# Autodesk Inventor assembly: y-axis
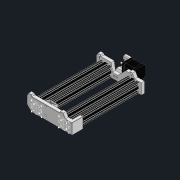
[picture p0: Inventor's stored thumbnail of the model, 180x180]
Saved by Autodesk Inventor 2021 (Build 250183000, 183)
## iProperties
Created: 2021-03-09
Part Number: y-axis
Document SubType Name: Assembly
Designer: Alex
Author: Alex
## Documents named in this file (7)
- C:\Users\arbra\OneDrive\Documents\3D Printer\IPT\ASSEMBLY\y-axis.iam
- C:\Users\arbra\OneDrive\Documents\3D Printer\IPT\PARTS\Y-AXIS\y-front-V2.ipt
- C:\Users\arbra\OneDrive\Documents\3D Printer\IPT\PARTS\Y-AXIS\y-idler-V2.ipt
- C:\Users\arbra\OneDrive\Documents\3D Printer\IPT\PARTS\MECHANICAL\V-Slot 40x40x500 Linear Rail.ipt
- C:\Users\arbra\OneDrive\Documents\3D Printer\IPT\PARTS\Y-AXIS\y-rear-V2.ipt
- C:\Users\arbra\OneDrive\Documents\3D Printer\IPT\PARTS\Y-AXIS\y-stepper-mount.ipt
- C:\Users\arbra\OneDrive\Documents\3D Printer\IPT\PARTS\MECHANICAL\Nema 17 Stepper Motor.ipt
## Components (7 placed, 6 different names)
1. y-front-V2:1 — Insert:1, Insert:2, Insert:3, Insert:4, Insert:5, Insert:6
2. y-idler-V2:1 — Insert:1, Insert:2
3. V-Slot Linear Rail:1 — Insert:3, Insert:4, Insert:7, Insert:8
4. V-Slot Linear Rail:2 — Insert:5, Insert:6, Insert:9, Insert:10
5. y-rear-V2:1 — Insert:7, Insert:8, Insert:9, Insert:10, Insert:11, Insert:12
6. y-stepper-mount:1 — Insert:11, Insert:12, Insert:13, Insert:14
7. Nema 17 Stepper Motor:1 — Insert:13, Insert:14
## Relationships (14: Insert 14)
- Insert:1: y-front-V2:1 ↔ y-idler-V2:1
- Insert:2: y-front-V2:1 ↔ y-idler-V2:1
- Insert:3: y-front-V2:1 ↔ V-Slot Linear Rail:1
- Insert:4: y-front-V2:1 ↔ V-Slot Linear Rail:1
- Insert:5: y-front-V2:1 ↔ V-Slot Linear Rail:2
- Insert:6: y-front-V2:1 ↔ V-Slot Linear Rail:2
- Insert:7: V-Slot Linear Rail:1 ↔ y-rear-V2:1
- Insert:8: V-Slot Linear Rail:1 ↔ y-rear-V2:1
- Insert:9: V-Slot Linear Rail:2 ↔ y-rear-V2:1
- Insert:10: V-Slot Linear Rail:2 ↔ y-rear-V2:1
- Insert:11: y-rear-V2:1 ↔ y-stepper-mount:1
- Insert:12: y-rear-V2:1 ↔ y-stepper-mount:1
- Insert:13: y-stepper-mount:1 ↔ Nema 17 Stepper Motor:1
- Insert:14: y-stepper-mount:1 ↔ Nema 17 Stepper Motor:1
